# Autodesk Inventor assembly: test-model-2025stp
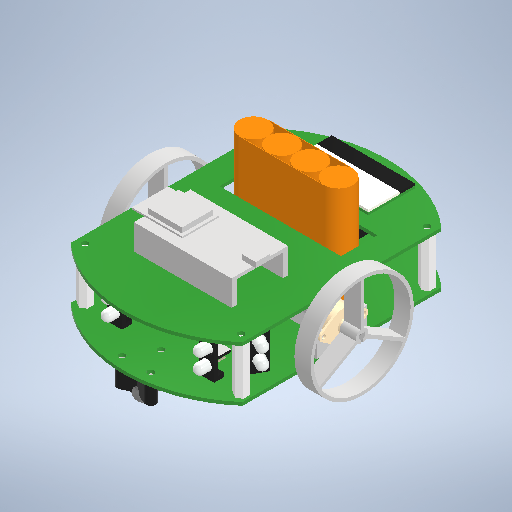
[picture p0: Inventor's stored thumbnail of the model, 512x512]
Saved by Autodesk Inventor 2025.3 (Build 293356000, 356)
## iProperties
Created: 2025-05-29
Part Number: test-model-2025stp
Document SubType Name: Assembly
Designer: yamashita1
Author: yamashita1
## Documents named in this file (11)
- G:\マイドライブ\project\micro-mouse\3D-Model\test-model-2025stp.iam
- G:\マイドライブ\project\micro-mouse\3D-Model\BaseBoard2.ipt
- G:\マイドライブ\project\micro-mouse\3D-Model\BallCaster-H16.ipt
- G:\マイドライブ\project\micro-mouse\3D-Model\Photo-Sensor.iam
- G:\マイドライブ\project\micro-mouse\3D-Model\Spacer-M3H24.ipt
- G:\マイドライブ\project\micro-mouse\3D-Model\ESP32-DevKitC.ipt
- G:\マイドライブ\project\micro-mouse\3D-Model\NiMH-Battery.ipt
- G:\マイドライブ\project\micro-mouse\3D-Model\BaseBoard2B.ipt
- G:\マイドライブ\project\micro-mouse\3D-Model\AQM1602Y.ipt
- G:\マイドライブ\project\micro-mouse\3D-Model\Stepper-D15-S18_asm.iam
- G:\マイドライブ\project\micro-mouse\3D-Model\D-Shaft_Wheel4.ipt
## Components (20 placed, 10 different names)
1. BaseBoard2:1 — メイト:7, メイト:8, メイト:9, メイト:18, メイト:19, メイト:20, メイト:21, メイト:22, メイト:23, メイト:24, メイト:25, メイト:26, メイト:27, メイト:28, メイト:29, メイト:30, メイト:36, メイト:38, メイト:39, メイト:40, メイト:41, メイト:42, メイト:43, メイト:46, メイト:47, メイト:48
2. BallCaster-H16:1 — メイト:7, メイト:8, メイト:9
3. Photo-Sensor:1 [sub-assembly] — メイト:18
4. Photo-Sensor:2 [sub-assembly] — メイト:19
5. Photo-Sensor:3 [sub-assembly] — メイト:20
6. Photo-Sensor:4 [sub-assembly] — メイト:21
7. Photo-Sensor:5 [sub-assembly] — メイト:22
8. Spacer-M3H24:1 — メイト:23, メイト:29
9. Spacer-M3H24:2 — メイト:24, メイト:30, メイト:31, メイト:32
10. Spacer-M3H24:3 — メイト:25, メイト:27, メイト:33
11. Spacer-M3H24:4 — メイト:26, メイト:28
12. ESP32-DevKitC:1 — メイト:35
13. BaseBoard2B:1 — メイト:31, メイト:32, メイト:33, メイト:35, メイト:37
14. NiMH-Battery:1 — メイト:36
15. AQM1602Y:1 — メイト:37
16. Stepper-D15-S18_asm:1 [sub-assembly] — メイト:39, メイト:42, メイト:43, メイト:45, フラッシュ:2
17. Stepper-D15-S18_asm:2 [sub-assembly] — メイト:38, メイト:40, メイト:41, メイト:44, フラッシュ:1
18. D-Shaft_Wheel4:1 — メイト:44, フラッシュ:1
19. D-Shaft_Wheel4:2 — メイト:45, フラッシュ:2
20. BallCaster-H16:2 — メイト:46, メイト:47, メイト:48
## Relationships (35: Mate 33, Flush 2)
- メイト:7 [Mate]: BaseBoard2:1 ↔ BallCaster-H16:1
- メイト:8 [Mate]: BaseBoard2:1 ↔ BallCaster-H16:1
- メイト:9 [Mate]: BaseBoard2:1 ↔ BallCaster-H16:1
- メイト:18 [Mate]: BaseBoard2:1 ↔ Photo-Sensor:1
- メイト:19 [Mate]: BaseBoard2:1 ↔ Photo-Sensor:2
- メイト:20 [Mate]: BaseBoard2:1 ↔ Photo-Sensor:3
- メイト:21 [Mate]: BaseBoard2:1 ↔ Photo-Sensor:4
- メイト:22 [Mate]: BaseBoard2:1 ↔ Photo-Sensor:5
- メイト:23 [Mate]: BaseBoard2:1 ↔ Spacer-M3H24:1
- メイト:24 [Mate]: BaseBoard2:1 ↔ Spacer-M3H24:2
- メイト:25 [Mate]: BaseBoard2:1 ↔ Spacer-M3H24:3
- メイト:26 [Mate]: BaseBoard2:1 ↔ Spacer-M3H24:4
- メイト:27 [Mate]: BaseBoard2:1 ↔ Spacer-M3H24:3
- メイト:28 [Mate]: BaseBoard2:1 ↔ Spacer-M3H24:4
- メイト:29 [Mate]: BaseBoard2:1 ↔ Spacer-M3H24:1
- メイト:30 [Mate]: BaseBoard2:1 ↔ Spacer-M3H24:2
- メイト:31 [Mate]: Spacer-M3H24:2 ↔ BaseBoard2B:1
- メイト:32 [Mate]: Spacer-M3H24:2 ↔ BaseBoard2B:1
- メイト:33 [Mate]: Spacer-M3H24:3 ↔ BaseBoard2B:1
- メイト:35 [Mate]: ESP32-DevKitC:1 ↔ BaseBoard2B:1
- メイト:36 [Mate]: BaseBoard2:1 ↔ NiMH-Battery:1
- メイト:37 [Mate] (1 mm): BaseBoard2B:1 ↔ AQM1602Y:1
- メイト:38 [Mate]: BaseBoard2:1 ↔ Stepper-D15-S18_asm:2
- メイト:39 [Mate]: BaseBoard2:1 ↔ Stepper-D15-S18_asm:1
- メイト:40 [Mate]: BaseBoard2:1 ↔ Stepper-D15-S18_asm:2
- メイト:41 [Mate]: BaseBoard2:1 ↔ Stepper-D15-S18_asm:2
- メイト:42 [Mate]: BaseBoard2:1 ↔ Stepper-D15-S18_asm:1
- メイト:43 [Mate]: BaseBoard2:1 ↔ Stepper-D15-S18_asm:1
- メイト:44 [Mate]: Stepper-D15-S18_asm:2 ↔ D-Shaft_Wheel4:1
- フラッシュ:1 [Flush]: Stepper-D15-S18_asm:2 ↔ D-Shaft_Wheel4:1
- メイト:45 [Mate]: Stepper-D15-S18_asm:1 ↔ D-Shaft_Wheel4:2
- フラッシュ:2 [Flush]: Stepper-D15-S18_asm:1 ↔ D-Shaft_Wheel4:2
- メイト:46 [Mate]: BaseBoard2:1 ↔ BallCaster-H16:2
- メイト:47 [Mate]: BaseBoard2:1 ↔ BallCaster-H16:2
- メイト:48 [Mate]: BaseBoard2:1 ↔ BallCaster-H16:2
